# Autodesk Inventor assembly: iris
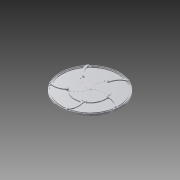
[picture p0: Inventor's stored thumbnail of the model, 180x180]
Saved by Autodesk Inventor 2015 (Build 190159000, 159)
## iProperties
Created: 2015-02-04
Part Number: iris
Document SubType Name: Assembly
Designer: janov_000
Author: janov_000
## Documents named in this file (5)
- C:\Users\janov_000\Documents\EiT iris\iris.iam
- C:\Users\janov_000\Documents\EiT iris\bakplate.ipt
- C:\Users\janov_000\Documents\EiT iris\ytterring.ipt
- C:\Users\janov_000\Documents\EiT iris\blad.ipt
- C:\Users\janov_000\Documents\EiT iris\ledeplate.ipt
## Components (12 placed, 4 different names)
1. bakplate:1 — Mate:2, Insert:1, Mate:3, Insert:2, Rotational:1, Insert:7, Insert:10, Insert:11
2. ytterring:1 — Flush:1, Insert:3, Rotational:1, Insert:6, Insert:9, Insert:12, Insert:13
3. blad:1 — Mate:2, Insert:1, Insert:4
4. blad:2 — Mate:3, Insert:2, Insert:5
5. ledeplate:1 — Flush:1, Insert:3, Insert:4
6. ledeplate:2 — Insert:5, Insert:6
7. blad:3 — Insert:7, Insert:8
8. ledeplate:3 — Insert:8, Insert:9
9. blad:4 — Insert:10, Insert:14
10. blad:5 — Insert:11, Insert:15
11. ledeplate:4 — Insert:12, Insert:14
12. ledeplate:5 — Insert:13, Insert:15
## Relationships (19: Insert 15, Mate 2, Flush 1, RevoluteJoint 1)
- Mate:2: bakplate:1 ↔ blad:1
- Insert:1: bakplate:1 ↔ blad:1
- Mate:3: bakplate:1 ↔ blad:2
- Insert:2: bakplate:1 ↔ blad:2
- Flush:1: ytterring:1 ↔ ledeplate:1
- Insert:3: ytterring:1 ↔ ledeplate:1
- Insert:4: blad:1 ↔ ledeplate:1
- Rotational:1 [RevoluteJoint]: bakplate:1 ↔ ytterring:1
- Insert:5: blad:2 ↔ ledeplate:2
- Insert:6: ytterring:1 ↔ ledeplate:2
- Insert:7: bakplate:1 ↔ blad:3
- Insert:8: blad:3 ↔ ledeplate:3
- Insert:9: ytterring:1 ↔ ledeplate:3
- Insert:10: bakplate:1 ↔ blad:4
- Insert:11: bakplate:1 ↔ blad:5
- Insert:12: ytterring:1 ↔ ledeplate:4
- Insert:13: ytterring:1 ↔ ledeplate:5
- Insert:14: blad:4 ↔ ledeplate:4
- Insert:15: blad:5 ↔ ledeplate:5
